# Autodesk Inventor assembly: Right-Brush
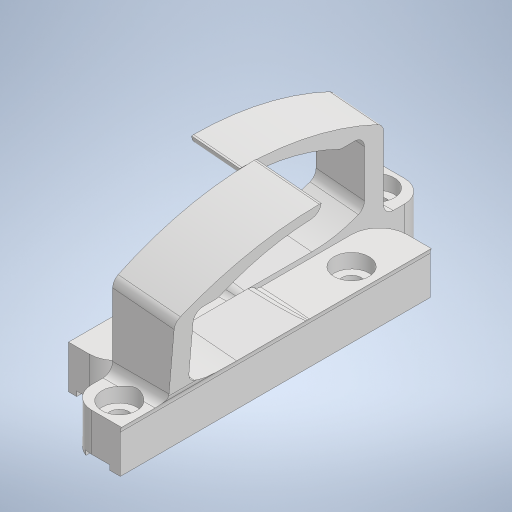
[picture p0: Inventor's stored thumbnail of the model, 512x512]
Saved by Autodesk Inventor 2024 (Build 280153000, 153)
## iProperties
Created: 2023-12-18
Part Number: Right-Brush
Document SubType Name: Assembly
Designer: shaun
Author: shaun
## Documents named in this file (3)
- Z:\VirtualBox VMs\Baxter\ROS2-Baxter\3D Models\Gripper V2\Left-Dustpan.iam
- Z:\VirtualBox VMs\Baxter\ROS2-Baxter\3D Models\Gripper V2\Left-Dustpan-Bottom.ipt
- Z:\VirtualBox VMs\Baxter\ROS2-Baxter\3D Models\Gripper V2\Left-Dustpan-Top.ipt
## Components (2 placed, 2 different names)
1. Left-Dustpan-Top:1 — Mate:1, Mate:2, Mate:3, Flush:1
2. Left-Dustpan-Bottom:1 — Mate:3, Flush:1
## Relationships (4: Mate 3, Flush 1)
- Mate:1: Left-Dustpan-Top:1
- Mate:2: Left-Dustpan-Top:1
- Mate:3: Left-Dustpan-Top:1 ↔ Left-Dustpan-Bottom:1
- Flush:1: Left-Dustpan-Top:1 ↔ Left-Dustpan-Bottom:1
